# Autodesk Inventor assembly: outer
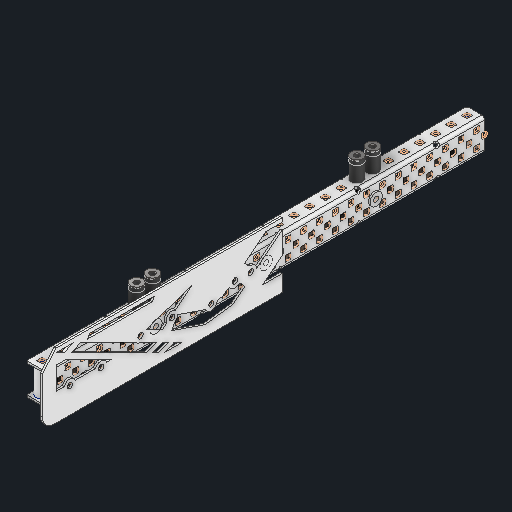
[picture p0: Inventor's stored thumbnail of the model, 512x512]
Saved by Autodesk Inventor 2024 (Build 280153000, 153)
## iProperties
Created: 2023-10-29
Part Number: outer
Document SubType Name: Assembly
Designer: Averey Ku
Author: Averey Ku
## Documents named in this file (15)
- C:\Users\avere\Documents\rbp_cad\zoomba_v0.1\chassis\drivebay\outer.iam
- C:\Users\avere\Documents\rbp_cad\VEX-CAD-Inventor-1.41\Motion\Insert Circle.ipt
- C:\Users\avere\Documents\rbp_cad\VEX-CAD-Inventor-1.41\Structure\C Channel\Aluminum 1x2x1\Alu C 1x2x1x28.ipt
- C:\Users\avere\Documents\rbp_cad\hardware\.375 OD Aluminum Spacer 0.875.ipt
- C:\Users\avere\Documents\rbp_cad\VEX-CAD-Inventor-1.41\Motion\Spacers\Spacer Nylon .375 OD.ipt
- C:\Users\avere\Documents\rbp_cad\VEX-CAD-Inventor-1.41\Motion\Spacers\Spacer Nylon .375 OD\NSpacer .375 OD x .500.ipt
- C:\Users\avere\Documents\rbp_cad\zoomba_v0.1\chassis\drivebay\custom_parts\washer_thick.ipt
- C:\Users\avere\Documents\rbp_cad\VEX-CAD-Inventor-1.41\Motion\Spacers\Spacer Nylon .500 OD\NSpacer White .500 OD x .250.ipt
- C:\Users\avere\Documents\rbp_cad\VEX-CAD-Inventor-1.41\Motion\Spacers\Spacer Nylon .500 OD.ipt
- C:\Users\avere\Documents\rbp_cad\VEX-CAD-Inventor-1.41\Structure\Standoff\Standoff .875.ipt
- C:\Users\avere\Documents\rbp_cad\VEX-CAD-Inventor-1.41\Structure\Standoff.ipt
- C:\Users\avere\Documents\rbp_cad\zoomba_v0.1\chassis\drivebay\custom_parts\sideplate.ipt
- C:\Users\avere\Documents\rbp_cad\VEX-CAD-Inventor-1.41\Motion\Spacers\Washer Steel\SWasher .375 OD x .031250.ipt
- C:\Users\avere\Documents\rbp_cad\VEX-CAD-Inventor-1.41\Motion\Spacers\Washer Steel.ipt
- C:\Users\avere\Documents\rbp_cad\VEX-CAD-Inventor-1.41\Motion\Spacers\Spacer Nylon .375 OD\NSpacer .375 OD x .125.ipt
## Components (26 placed, 10 different names)
1. Insert Circle:2 — Insert:2
2. Insert Circle:4 — Insert:4
3. Insert Circle:6 — Insert:6
4. Alu C 1x2x1x28:1 — Insert:2, Insert:4, Insert:6, Insert:8, Insert:17, Insert:23, Insert:24, Insert:25, Insert:26, Insert:27, Insert:28, Insert:29, Mate:1, Insert:34, Insert:35, Insert:36, Insert:37
5. .375 OD Aluminum Spacer 0.875:1 — Insert:8
6. washer_thick:1 — Insert:17, Insert:18
7. NSpacer White .500 OD x .250:1 — Insert:18
8. Standoff .875:1 — Insert:24
9. Standoff .875:2 — Insert:23
10. Standoff .875:3 — Insert:25
11. Standoff .875:4 — Insert:27
12. Standoff .875:5 — Insert:26
13. .375 OD Aluminum Spacer 0.875:2 — Insert:28
14. sideplate:1 — Insert:29, Mate:1
15. SWasher .375 OD x .031250:1
16. NSpacer .375 OD x .500:13 — Insert:34
17. NSpacer .375 OD x .125:14
18. SWasher .375 OD x .031250:2
19. NSpacer .375 OD x .500:15 — Insert:35
20. NSpacer .375 OD x .125:16
21. NSpacer .375 OD x .500:17 — Insert:36, Insert:38
22. NSpacer .375 OD x .125:18 — Insert:38, Insert:41
23. SWasher .375 OD x .031250:3 — Insert:41
24. NSpacer .375 OD x .500:19 — Insert:37, Insert:39
25. NSpacer .375 OD x .125:20 — Insert:39, Insert:40
26. SWasher .375 OD x .031250:4 — Insert:40
## Relationships (26: Insert 25, Mate 1)
- Insert:2: Insert Circle:2 ↔ Alu C 1x2x1x28:1
- Insert:4: Insert Circle:4 ↔ Alu C 1x2x1x28:1
- Insert:6: Insert Circle:6 ↔ Alu C 1x2x1x28:1
- Insert:8: Alu C 1x2x1x28:1 ↔ .375 OD Aluminum Spacer 0.875:1
- Insert:17: Alu C 1x2x1x28:1 ↔ washer_thick:1
- Insert:18: washer_thick:1 ↔ NSpacer White .500 OD x .250:1
- Insert:23: Alu C 1x2x1x28:1 ↔ Standoff .875:2
- Insert:24: Alu C 1x2x1x28:1 ↔ Standoff .875:1
- Insert:25: Alu C 1x2x1x28:1 ↔ Standoff .875:3
- Insert:26: Alu C 1x2x1x28:1 ↔ Standoff .875:5
- Insert:27: Alu C 1x2x1x28:1 ↔ Standoff .875:4
- Insert:28: Alu C 1x2x1x28:1 ↔ .375 OD Aluminum Spacer 0.875:2
- Insert:29: Alu C 1x2x1x28:1 ↔ sideplate:1
- Mate:1: Alu C 1x2x1x28:1 ↔ sideplate:1
- [Insert]: NSpacer .375 OD x .500:13 ↔ NSpacer .375 OD x .125:14
- [Insert]: SWasher .375 OD x .031250:1 ↔ NSpacer .375 OD x .125:14
- [Insert]: NSpacer .375 OD x .500:15 ↔ NSpacer .375 OD x .125:16
- [Insert]: SWasher .375 OD x .031250:2 ↔ NSpacer .375 OD x .125:16
- Insert:34: Alu C 1x2x1x28:1 ↔ NSpacer .375 OD x .500:13
- Insert:35: Alu C 1x2x1x28:1 ↔ NSpacer .375 OD x .500:15
- Insert:36: Alu C 1x2x1x28:1 ↔ NSpacer .375 OD x .500:17
- Insert:37: Alu C 1x2x1x28:1 ↔ NSpacer .375 OD x .500:19
- Insert:38: NSpacer .375 OD x .500:17 ↔ NSpacer .375 OD x .125:18
- Insert:39: NSpacer .375 OD x .500:19 ↔ NSpacer .375 OD x .125:20
- Insert:40: NSpacer .375 OD x .125:20 ↔ SWasher .375 OD x .031250:4
- Insert:41: NSpacer .375 OD x .125:18 ↔ SWasher .375 OD x .031250:3
## Named parameters: d60_d242 = 0 mm, d61_d243 = 0 mm
